# Autodesk Inventor assembly: assemble
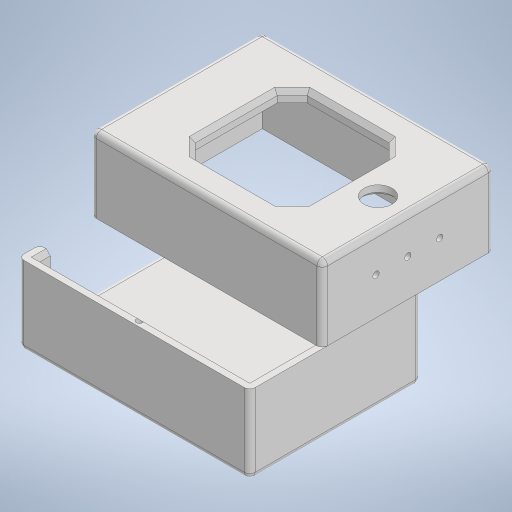
[picture p0: Inventor's stored thumbnail of the model, 512x512]
Saved by Autodesk Inventor 2024 (Build 280153000, 153)
## iProperties
Created: 2024-03-11
Part Number: assemble
Document SubType Name: Assembly
Designer: SSAFY
Author: SSAFY
## Documents named in this file (3)
- C:\Users\SSAFY\Desktop\TIL\3D\3D\assemble.iam
- C:\Users\SSAFY\Desktop\TIL\3D\3D\housing_bottom.ipt
- C:\Users\SSAFY\Desktop\TIL\3D\3D\housing_top.ipt
## Components (2 placed, 2 different names)
1. housing_bottom:2 — 플러쉬:1, 플러쉬:2, 플러쉬:3, 메이트:1, 플러쉬:6
2. housing_top:2 — 메이트:1, 플러쉬:6
## Relationships (5: Flush 4, Mate 1)
- 플러쉬:1 [Flush]: housing_bottom:2
- 플러쉬:2 [Flush]: housing_bottom:2
- 플러쉬:3 [Flush]: housing_bottom:2
- 메이트:1 [Mate]: housing_bottom:2 ↔ housing_top:2
- 플러쉬:6 [Flush]: housing_bottom:2 ↔ housing_top:2
